# Autodesk Inventor assembly: ThumbAssembly
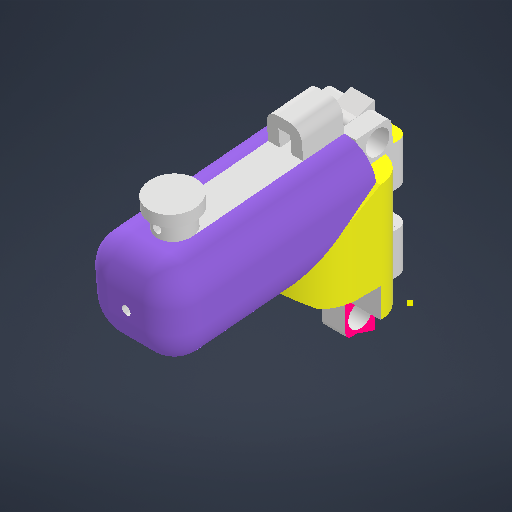
[picture p0: Inventor's stored thumbnail of the model, 512x512]
Saved by Autodesk Inventor 2026 (Build 300175050, 175E)
## iProperties
Created: 2026-06-23
Part Number: ThumbAssembly
Document SubType Name: Assembly
Designer: SaiAn
Author: SaiAn
## Documents named in this file (3)
- C:\EMG Biomechanical Arm\ThumbAssembly.iam
- C:\EMG Biomechanical Arm\FingerTopThumb.ipt
- C:\EMG Biomechanical Arm\FingerMiddleThumb.ipt
## Components (2 placed, 2 different names)
1. FingerTopThumb:1 — Mate:1, Mate:2
2. FingerMiddleThumb:1 — Mate:1, Mate:2
## Relationships (2: Mate 2)
- Mate:1: FingerTopThumb:1 ↔ FingerMiddleThumb:1
- Mate:2: FingerTopThumb:1 ↔ FingerMiddleThumb:1
